# Autodesk Inventor assembly: Rail truck area subassembly v2
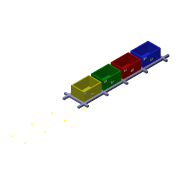
[picture p0: Inventor's stored thumbnail of the model, 180x180]
Saved by Autodesk Inventor 2015 (Build 190159000, 159)
## iProperties
Created: 2015-04-10
Part Number: Rail truck area subassembly v2
Document SubType Name: Assembly
Designer: Vukica
Author: Vukica
## Documents named in this file (6)
- D:\Dropbox\Dropbox\Service\IEEE\!Final Rules\2016Hardware_Court_v8-aug12\Rail truck area subassembly v2.iam
- D:\Dropbox\Dropbox\Service\IEEE\!Final Rules\2016Hardware_Court_v8-aug12\Rail zone.ipt
- D:\Dropbox\Dropbox\Service\IEEE\!Final Rules\2016Hardware_Court_v8-aug12\Bucket.ipt
- D:\Dropbox\Dropbox\Service\IEEE\!Final Rules\2016Hardware_Court_v8-aug12\Bucket green.ipt
- D:\Dropbox\Dropbox\Service\IEEE\!Final Rules\2016Hardware_Court_v8-aug12\Bucket yellow.ipt
- D:\Dropbox\Dropbox\Service\IEEE\!Final Rules\2016Hardware_Court_v8-aug12\Bucket red.ipt
## Components (5 placed, 5 different names)
1. Rail zone:1 — Flush:1, Mate:1, Mate:2, Mate:3
2. Bucket:1 — Flush:1, Flush:2, Flush:3, Flush:4, Flush:5
3. Bucket green:1 — Flush:4, Flush:6, Mate:2
4. Bucket yellow:1 — Flush:2, Flush:5, Flush:6, Flush:7, Mate:3
5. Bucket red:1 — Flush:3, Flush:7, Mate:1
## Relationships (10: Flush 7, Mate 3)
- Flush:1: Rail zone:1 ↔ Bucket:1
- Flush:2: Bucket:1 ↔ Bucket yellow:1
- Flush:3: Bucket:1 ↔ Bucket red:1
- Flush:4: Bucket:1 ↔ Bucket green:1
- Flush:5: Bucket:1 ↔ Bucket yellow:1
- Flush:6: Bucket green:1 ↔ Bucket yellow:1
- Flush:7: Bucket yellow:1 ↔ Bucket red:1
- Mate:1 (3.175 mm): Rail zone:1 ↔ Bucket red:1
- Mate:2 (3.175 mm): Rail zone:1 ↔ Bucket green:1
- Mate:3 (3.175 mm): Rail zone:1 ↔ Bucket yellow:1
